# Autodesk Inventor assembly: structure
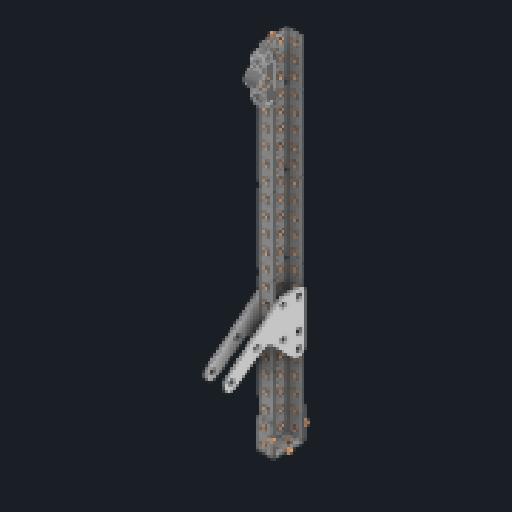
[picture p0: Inventor's stored thumbnail of the model, 512x512]
Saved by Autodesk Inventor 2025 (Build 290162000, 162)
## iProperties
Created: 2024-10-13
Part Number: structure
Document SubType Name: Assembly
Designer: Averey Ku
Author: Averey Ku
## Documents named in this file (5)
- D:\vex_robotics_high_stakes\hardware\cad\bots\high_stakes_v2\tower\structure\vertical.iam
- D:\vex_robotics_high_stakes\hardware\cad\robpros_cad_lib\Structure\C Channel\Aluminum 2x2x2\Alu C 2x2x2x1.ipt
- D:\vex_robotics_high_stakes\hardware\cad\robpros_cad_lib\Structure\C Channel\Aluminum 1x2x1\Alu C 1x2x1x23.ipt
- D:\vex_robotics_high_stakes\hardware\cad\robpros_cad_lib\Motion\Shaft HS\HS Pillow Bearing Block.ipt
- D:\vex_robotics_high_stakes\hardware\cad\bots\high_stakes_v2\tower\structure\custom_parts\triangle_brace_gusset.ipt
## Components (5 placed, 4 different names)
1. Alu C 2x2x2x1:1 — Mate:2
2. Alu C 1x2x1x23:1 — Insert:4, Mate:5, Insert:6, Mate:7, Insert:7, Mate:8
3. HS Pillow Bearing Block:1 — Insert:4, Mate:5
4. triangle_brace_gusset:1 — Insert:6, Mate:7
5. triangle_brace_gusset:2 — Insert:7, Mate:8
## Relationships (9: Mate 5, Insert 4)
- [Insert]: Alu C 2x2x2x1:1 ↔ Alu C 1x2x1x23:1
- [Mate]: Alu C 2x2x2x1:1 ↔ Alu C 1x2x1x23:1
- Mate:2: Alu C 2x2x2x1:1
- Insert:4: Alu C 1x2x1x23:1 ↔ HS Pillow Bearing Block:1
- Mate:5: Alu C 1x2x1x23:1 ↔ HS Pillow Bearing Block:1
- Insert:6: Alu C 1x2x1x23:1 ↔ triangle_brace_gusset:1
- Mate:7: Alu C 1x2x1x23:1 ↔ triangle_brace_gusset:1
- Insert:7 (12.7 mm): Alu C 1x2x1x23:1 ↔ triangle_brace_gusset:2
- Mate:8: Alu C 1x2x1x23:1 ↔ triangle_brace_gusset:2
